# Autodesk Inventor assembly: forkMountForDecTripV03
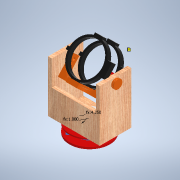
[picture p0: Inventor's stored thumbnail of the model, 180x180]
Saved by Autodesk Inventor 2022.2 (Build 262287010, 287A)
## iProperties
Created: 2020-11-06
Part Number: forkMountForDecTripV03
Document SubType Name: Assembly
Designer: robst
Mass: 6772.5 g
Surface Area: 8494.13 cm^2
Volume: 2840.29 cm^3
Density: 2.38444 g/cm^3
Author: robst
## Documents named in this file (13)
- C:\git\CAD-Development\robSteele\ShapeWays\TelescopeProjects\TelescopeMountNov2020\forkMountForDecTripV03.iam
- C:\git\CAD-Development\robSteele\ShapeWays\TelescopeProjects\TelescopeMount\telescopeTube.ipt
- C:\git\CAD-Development\robSteele\ShapeWays\TelescopeProjects\TelescopeMount\celestronTubeBracket.ipt
- C:\git\CAD-Development\robSteele\ShapeWays\TelescopeProjects\TelescopeMountNov2020\connectorToTubeBrackeCradle.ipt
- C:\git\CAD-Development\robSteele\ShapeWays\TelescopeProjects\TelescopeMountNov2020\hexBushingForConnectorPiece.ipt
- C:\git\CAD-Development\robSteele\ShapeWays\TelescopeProjects\TelescopeMountNov2020\forkBaseWithWormGearAndLock.iam
- C:\git\CAD-Development\robSteele\ShapeWays\TelescopeProjects\TelescopeMountNov2020\attachementToTripodWithInserts.iam
- C:\Users\robst\Documents\Inventor\Content Center Files\R2021\en-US\ANSI B18.22.1\ANSI B18.22.1 - No. 10 - Type A.ipt
- C:\Users\robst\Documents\Inventor\Content Center Files\R2021\en-US\U UNC 2605\Unbrako - 10 x 5_8 - 24(10).ipt
- C:\git\CAD-Development\robSteele\ShapeWays\TelescopeProjects\TelescopeMountNov2020\1_2x1_2-hexBearing.ipt
- c:\git\CAD-MfgResources\McMaster-Carr\Screw\92949A153_6_32x1-18-8 Stainless Steel Button Head Hex Drive Screw.ipt
- C:\git\CAD-Development\robSteele\ShapeWays\TelescopeProjects\TelescopeMount\woodForkAssembly02.ipt
- C:\git\CAD-Development\robSteele\ShapeWays\TelescopeProjects\TelescopeMountNov2020\connectForkToHexShaft.ipt
## Components (23 placed, 12 different names)
1. telescopeTube:1 — Insert:1
2. connectorToTubeBrackeCradle:1 — Mate:10, Mate:11, Mate:12, Mate:13, Mate:14, Mate:15, Mate:23, Mate:26, Mate:27
3. celestronTubeBracket:1 — Insert:1, Mate:13, Mate:14, Mate:15
4. celestronTubeBracket:2 — Mate:10, Mate:11, Mate:12
5. woodForkAssembly02:2 — Insert:10, Mate:34, Insert:11, Insert:12
6. hexBushingForConnectorPiece:1 — Mate:23, Mate:26, Mate:27, Insert:11
7. forkBaseWithWormGearAndLock:1 [sub-assembly] — Mate:32, Mate:33, Insert:9, Insert:10
8. attachementToTripodWithInserts:1 [sub-assembly] — Insert:9
9. 1_2x1_2-hexBearing:1
10. 92949A153_6_32x1-18-8 Stainless Steel Button Head Hex Drive Screw:1
11. connectForkToHexShaft:1 — Mate:34, Insert:12
12. Unbrako UNC Hex Socket Button Cap - Inch 10 x 5/8:1 — Insert:5
13. Plain Washer (Inch) No. 10 - Type A:1 — Mate:32, Mate:33, Insert:5
14. Unbrako UNC Hex Socket Button Cap - Inch 10 x 5/8:2
15. Plain Washer (Inch) No. 10 - Type A:2
16. Unbrako UNC Hex Socket Button Cap - Inch 10 x 5/8:3
17. Plain Washer (Inch) No. 10 - Type A:3
18. Unbrako UNC Hex Socket Button Cap - Inch 10 x 5/8:4
19. Plain Washer (Inch) No. 10 - Type A:4
20. Unbrako UNC Hex Socket Button Cap - Inch 10 x 5/8:5
21. Plain Washer (Inch) No. 10 - Type A:5
22. Unbrako UNC Hex Socket Button Cap - Inch 10 x 5/8:6
23. Plain Washer (Inch) No. 10 - Type A:6
## Component patterns: (6 elements, first: Unbrako UNC Hex Socket Button Cap - Inch 10 x 5/8:1 + Plain Washer (Inch) No. 10 - Type A:1)
## Relationships (21: Mate 13, Insert 6, Flush 2)
- Insert:1 (203.2 mm): telescopeTube:1 ↔ celestronTubeBracket:1
- Mate:10: connectorToTubeBrackeCradle:1 ↔ celestronTubeBracket:2
- Mate:11: connectorToTubeBrackeCradle:1 ↔ celestronTubeBracket:2
- Mate:12: connectorToTubeBrackeCradle:1 ↔ celestronTubeBracket:2
- Mate:13: connectorToTubeBrackeCradle:1 ↔ celestronTubeBracket:1
- Mate:14: connectorToTubeBrackeCradle:1 ↔ celestronTubeBracket:1
- Mate:15: connectorToTubeBrackeCradle:1 ↔ celestronTubeBracket:1
- [Flush]: woodForkAssembly02:2
- [Flush]: woodForkAssembly02:2
- Mate:23 (6.35 mm): connectorToTubeBrackeCradle:1 ↔ hexBushingForConnectorPiece:1
- Mate:26: connectorToTubeBrackeCradle:1 ↔ hexBushingForConnectorPiece:1
- Mate:27: connectorToTubeBrackeCradle:1 ↔ hexBushingForConnectorPiece:1
- [Mate]: woodForkAssembly02:2 ↔ forkBaseWithWormGearAndLock:1
- Mate:32: forkBaseWithWormGearAndLock:1 ↔ Plain Washer (Inch) No. 10 - Type A:1
- Mate:33: forkBaseWithWormGearAndLock:1 ↔ Plain Washer (Inch) No. 10 - Type A:1
- Insert:5: Unbrako UNC Hex Socket Button Cap - Inch 10 x 5/8:1 ↔ Plain Washer (Inch) No. 10 - Type A:1
- Insert:9: forkBaseWithWormGearAndLock:1 ↔ attachementToTripodWithInserts:1
- Insert:10: woodForkAssembly02:2 ↔ forkBaseWithWormGearAndLock:1
- Mate:34: woodForkAssembly02:2 ↔ connectForkToHexShaft:1
- Insert:11: woodForkAssembly02:2 ↔ hexBushingForConnectorPiece:1
- Insert:12: woodForkAssembly02:2 ↔ connectForkToHexShaft:1
